# Autodesk Inventor assembly: Apparatus Assembly V2
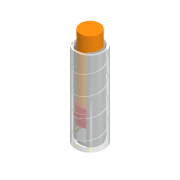
[picture p0: Inventor's stored thumbnail of the model, 180x180]
Saved by Autodesk Inventor 2020.4 (Build 244396000, 396)
## iProperties
Created: 2022-05-29
Part Number: Apparatus Assembly V2
Document SubType Name: Assembly
Designer: david
Author: david
## Documents named in this file (5)
- C:\Users\david\Desktop\ChalkBot\Apparatus Assembly V2.iam
- C:\Users\david\Desktop\ChalkBot\Chalk Holder.ipt
- C:\Users\david\Desktop\ChalkBot\Screw.ipt
- C:\Users\david\Desktop\ChalkBot\Sheath.ipt
- C:\Users\david\Desktop\ChalkBot\Chalk.ipt
## Components (4 placed, 4 different names)
1. Chalk Holder:1 — Cylindrical:1, Mate:1
2. Screw:1 — Cylindrical:1, Rotational:1
3. Sheath:1 — Rotational:1
4. Chalk:1 — Mate:1
## Relationships (3: CylindricalJoint 1, RevoluteJoint 1, Mate 1)
- Cylindrical:1: Chalk Holder:1 ↔ Screw:1
- Rotational:1 [RevoluteJoint]: Screw:1 ↔ Sheath:1
- Mate:1: Chalk Holder:1 ↔ Chalk:1
